# Autodesk Inventor assembly: Assembly
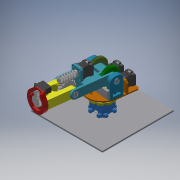
[picture p0: Inventor's stored thumbnail of the model, 180x180]
Saved by Autodesk Inventor 2019 (Build 230136000, 136)
## iProperties
Created: 2019-12-22
Part Number: Assembly
Material: Типовые
Document SubType Name: Assembly
Designer: Петров Иван
Author: Петров Иван
## Documents named in this file (3)
- E:\IVAN\Ivan_desktop\GitHub\Arm_manip\hardware\Assembly.iam
- E:\IVAN\Ivan_desktop\GitHub\Arm_manip\hardware\Assembly_floor.ipt
- E:\IVAN\Ivan_desktop\GitHub\Arm_manip\hardware\motor_holder_assembly.iam
## Components (2 placed, 2 different names)
1. Assembly_floor:1 — Совмещение:1, Совмещение:2, Совмещение:3
2. motor_holder_assembly:1 [sub-assembly] — Совмещение:1, Совмещение:2, Совмещение:3
## Relationships (3: Mate 3)
- Совмещение:1 [Mate]: Assembly_floor:1 ↔ motor_holder_assembly:1
- Совмещение:2 [Mate]: Assembly_floor:1 ↔ motor_holder_assembly:1
- Совмещение:3 [Mate]: Assembly_floor:1 ↔ motor_holder_assembly:1
